# Autodesk Inventor assembly: Zonnepaneel V1.0
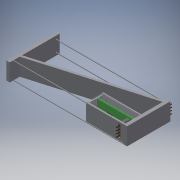
[picture p0: Inventor's stored thumbnail of the model, 180x180]
Saved by Autodesk Inventor 2018.3 (Build 223284000, 284)
## iProperties
Created: 2020-11-12
Part Number: Zonnepaneel V1.0
Document SubType Name: Assembly
Designer: daanv
Author: daanv
## Documents named in this file (4)
- C:\Users\daanv\OneDrive\Documenten\Life\Avans Project RED\Token\Zonnepaneel\V1.0\Zonnepaneel V1.0.iam
- C:\Users\daanv\OneDrive\Documenten\Life\Avans Project RED\Token\Zonnepaneel\V1.0\Zonnepaneel V1.0.ipt
- C:\Users\daanv\OneDrive\Documenten\Life\Avans Project RED\Token\Design 2\4pin male and female.ipt
- C:\Users\daanv\OneDrive\Documenten\Life\Avans Project RED\Token\Design 2\Token design 2.iam
## Components (3 placed, 3 different names)
1. Zonnepaneel V1.0:1 — Mate:1, Mate:2, Mate:3, Mate:5, Mate:6
2. 4pin male and female:2 — Mate:1, Mate:2, Mate:3
3. Token design 2:1 [sub-assembly] — Mate:5, Mate:6
## Relationships (5: Mate 5)
- Mate:1 (-8.5 mm): Zonnepaneel V1.0:1 ↔ 4pin male and female:2
- Mate:2: Zonnepaneel V1.0:1 ↔ 4pin male and female:2
- Mate:3: Zonnepaneel V1.0:1 ↔ 4pin male and female:2
- Mate:5: Zonnepaneel V1.0:1 ↔ Token design 2:1
- Mate:6: Zonnepaneel V1.0:1 ↔ Token design 2:1
